# Autodesk Inventor assembly: Assembly1
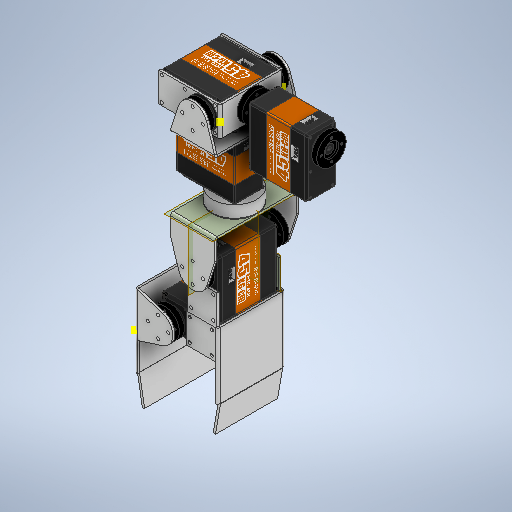
[picture p0: Inventor's stored thumbnail of the model, 512x512]
Saved by Autodesk Inventor 2025.2 (Build 292293000, 293)
## iProperties
Created: 2025-05-12
Part Number: Assembly1
Document SubType Name: Assembly
Designer: LG
Author: LG
## Documents named in this file (14)
- C:\Users\LG\Desktop\RHp_Humanoid_ver1\Assembly\6_right_Arm.iam
- C:\Users\LG\Desktop\RHp_Humanoid_ver1\Part\Frame\Arm\axis_19_top_frame.ipt
- C:\Users\LG\Desktop\RHp_Humanoid_ver1\Part\HTD-45H, Horn\HTD-45H\HTD-45H.ipt
- C:\Users\LG\Desktop\RHp_Humanoid_ver1\Part\HTD-45H, Horn\Horn\Top Horn.ipt
- C:\Users\LG\Desktop\RHp_Humanoid_ver1\Part\Frame\Arm\axis_4_top_frame.ipt
- C:\Users\LG\Desktop\RHp_Humanoid_ver1\Part\Frame\Arm\axis_21_bottom_frame.ipt
- C:\Users\LG\Desktop\RHp_Humanoid_ver1\Part\Frame\Arm\axis_22_top_frame(middle).ipt
- C:\Users\LG\Desktop\RHp_Humanoid_ver1\Part\Frame\Arm\axis_22_bottom_frame(middle).ipt
- C:\Users\LG\Desktop\RHp_Humanoid_ver1\Part\Frame\Arm\axis_24_bottom_frame.ipt
- C:\Users\LG\Desktop\RHp_Humanoid_ver1\Part\HTD-45H, Horn\Horn\Bottom Horn.ipt
- C:\Users\LG\Desktop\RHp_Humanoid_ver1\Part\Frame\Arm\axis_20_bottom_frame.ipt
- C:\Users\LG\Desktop\RHp_Humanoid_ver1\Part\Bolt, Bearing, Nut, Washer\2030 Teflon Sheet.ipt
- C:\Users\LG\Desktop\RHp_Humanoid_ver1\Part\HTD-45H, Horn\HTD-45H\HTD-45H.iam
- C:\Users\LG\Desktop\RHp_Humanoid_ver1\Part\Frame\Arm\axis_24_top_frame.ipt
## Components (23 placed, 12 different names)
1. Top Horn:3 — Mate:56, Mate:57, Mate:58, Mate:61
2. Bottom Horn:2 — Mate:54, Mate:55, Flush:31
3. HTD-45H:3 [sub-assembly] — Mate:54, Mate:55, Flush:31, Mate:56, Mate:57, Mate:58, Mate:59, Mate:60, Mate:62, Mate:63, Mate:64
4. axis_19_top_frame:1 — Flush:13, Flush:14, Mate:28, Mate:61, Mate:63, Mate:64
5. Bottom Horn:1 — Flush:28, Mate:41, Mate:42
6. Top Horn:2 — Mate:43, Mate:44, Mate:45, Mate:48
7. HTD-45H:1 — Flush:13, Flush:14, Mate:28, Flush:28, Mate:41, Mate:42, Mate:43, Mate:44, Mate:45, Mate:46, Mate:47, Flush:30
8. axis_20_bottom_frame:1 — Mate:46, Mate:47, Mate:48, Flush:29, Mate:49
9. HTD-45H:2 — Mate:13, Mate:14, Flush:4, Mate:15, Mate:17, Flush:29, Mate:49, Flush:30
10. axis_4_top_frame:1 — Mate:13, Mate:14, Flush:4, Mate:16, Flush:18, Mate:30, Mate:52
11. Top Horn:1 — Mate:15, Mate:16, Mate:17, Mate:50, Mate:51
12. 2030 Teflon Sheet:1 — Mate:50, Mate:51, Mate:52, Mate:53
13. axis_21_bottom_frame:1 — Flush:18, Mate:30, Mate:53, Mate:70, Mate:71, Mate:72, Mate:82
14. HTD-45H:4 [sub-assembly] — Mate:65, Mate:66, Flush:32, Mate:67, Mate:68, Mate:69, Mate:71, Mate:72, Mate:74, Mate:78, Flush:37, Flush:38, Flush:41
15. Bottom Horn:3 — Mate:65, Mate:66, Flush:32
16. Top Horn:4 — Mate:67, Mate:68, Mate:69, Mate:70
17. Top Horn:5 — Mate:77, Flush:35, Flush:36
18. Bottom Horn:4 — Mate:75, Mate:76, Flush:34, Mate:80
19. HTD-45H:5 [sub-assembly] — Mate:75, Mate:76, Flush:34, Mate:77, Flush:35, Flush:36, Mate:78, Flush:37, Flush:38, Mate:79, Mate:81, Flush:39, Flush:40, Mate:83, Mate:85, Flush:42
20. axis_22_top_frame(middle):1 — Flush:40, Flush:41, Mate:83, Mate:84
21. axis_22_bottom_frame(middle):1 — Mate:74, Flush:39, Mate:82
22. axis_24_bottom_frame:1 — Mate:79, Mate:80, Mate:81
23. axis_24_top_frame:1 — Mate:84, Mate:85, Flush:42
## Relationships (69: Mate 51, Flush 18)
- Mate:13: HTD-45H:2 ↔ axis_4_top_frame:1
- Mate:14: HTD-45H:2 ↔ axis_4_top_frame:1
- Flush:4: HTD-45H:2 ↔ axis_4_top_frame:1
- Mate:15: HTD-45H:2 ↔ Top Horn:1
- Mate:16: axis_4_top_frame:1 ↔ Top Horn:1
- Mate:17: HTD-45H:2 ↔ Top Horn:1
- Flush:13: axis_19_top_frame:1 ↔ HTD-45H:1
- Flush:14: axis_19_top_frame:1 ↔ HTD-45H:1
- Mate:28: axis_19_top_frame:1 ↔ HTD-45H:1
- Flush:18: axis_4_top_frame:1 ↔ axis_21_bottom_frame:1
- Mate:30: axis_4_top_frame:1 ↔ axis_21_bottom_frame:1
- Flush:28: Bottom Horn:1 ↔ HTD-45H:1
- Mate:41: Bottom Horn:1 ↔ HTD-45H:1
- Mate:42: Bottom Horn:1 ↔ HTD-45H:1
- Mate:43: Top Horn:2 ↔ HTD-45H:1
- Mate:44: Top Horn:2 ↔ HTD-45H:1
- Mate:45 (0.47 mm): Top Horn:2 ↔ HTD-45H:1
- Mate:46 (4.43 mm): HTD-45H:1 ↔ axis_20_bottom_frame:1
- Mate:47: HTD-45H:1 ↔ axis_20_bottom_frame:1
- Mate:48: Top Horn:2 ↔ axis_20_bottom_frame:1
- Flush:29: axis_20_bottom_frame:1 ↔ HTD-45H:2
- Mate:49: axis_20_bottom_frame:1 ↔ HTD-45H:2
- Flush:30: HTD-45H:1 ↔ HTD-45H:2
- Mate:50: Top Horn:1 ↔ 2030 Teflon Sheet:1
- Mate:51: Top Horn:1 ↔ 2030 Teflon Sheet:1
- Mate:52: axis_4_top_frame:1 ↔ 2030 Teflon Sheet:1
- Mate:53: 2030 Teflon Sheet:1 ↔ axis_21_bottom_frame:1
- Mate:54: Bottom Horn:2 ↔ HTD-45H:3
- Mate:55: Bottom Horn:2 ↔ HTD-45H:3
- Flush:31: Bottom Horn:2 ↔ HTD-45H:3
- Mate:56 (0.47 mm): Top Horn:3 ↔ HTD-45H:3
- Mate:57: Top Horn:3 ↔ HTD-45H:3
- Mate:58: Top Horn:3 ↔ HTD-45H:3
- Mate:59: HTD-45H:3
- Mate:60: HTD-45H:3
- Mate:61: Top Horn:3 ↔ axis_19_top_frame:1
- Mate:62: HTD-45H:3
- Mate:63: HTD-45H:3 ↔ axis_19_top_frame:1
- Mate:64: HTD-45H:3 ↔ axis_19_top_frame:1
- Mate:65: HTD-45H:4 ↔ Bottom Horn:3
- Mate:66: HTD-45H:4 ↔ Bottom Horn:3
- Flush:32: HTD-45H:4 ↔ Bottom Horn:3
- Mate:67 (0.47 mm): HTD-45H:4 ↔ Top Horn:4
- Mate:68: HTD-45H:4 ↔ Top Horn:4
- Mate:69: HTD-45H:4 ↔ Top Horn:4
- Mate:70: axis_21_bottom_frame:1 ↔ Top Horn:4
- Mate:71: axis_21_bottom_frame:1 ↔ HTD-45H:4
- Mate:72 (16.43 mm): axis_21_bottom_frame:1 ↔ HTD-45H:4
- Mate:74: HTD-45H:4 ↔ axis_22_bottom_frame(middle):1
- Mate:75: Bottom Horn:4 ↔ HTD-45H:5
- Mate:76: Bottom Horn:4 ↔ HTD-45H:5
- Flush:34: Bottom Horn:4 ↔ HTD-45H:5
- Mate:77 (0.47 mm): Top Horn:5 ↔ HTD-45H:5
- Flush:35: Top Horn:5 ↔ HTD-45H:5
- Flush:36: Top Horn:5 ↔ HTD-45H:5
- Mate:78: HTD-45H:4 ↔ HTD-45H:5
- Flush:37: HTD-45H:4 ↔ HTD-45H:5
- Flush:38: HTD-45H:4 ↔ HTD-45H:5
- Mate:79 (4.43 mm): HTD-45H:5 ↔ axis_24_bottom_frame:1
- Mate:80: Bottom Horn:4 ↔ axis_24_bottom_frame:1
- Mate:81 (10 mm): HTD-45H:5 ↔ axis_24_bottom_frame:1
- Flush:39: HTD-45H:5 ↔ axis_22_bottom_frame(middle):1
- Mate:82: axis_21_bottom_frame:1 ↔ axis_22_bottom_frame(middle):1
- Flush:40: HTD-45H:5 ↔ axis_22_top_frame(middle):1
- Flush:41: HTD-45H:4 ↔ axis_22_top_frame(middle):1
- Mate:83: HTD-45H:5 ↔ axis_22_top_frame(middle):1
- Mate:84: axis_22_top_frame(middle):1 ↔ axis_24_top_frame:1
- Mate:85: HTD-45H:5 ↔ axis_24_top_frame:1
- Flush:42: HTD-45H:5 ↔ axis_24_top_frame:1
